# Autodesk Inventor assembly: Drone_rotor_arm_assembly
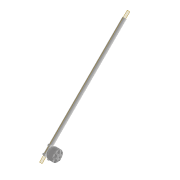
[picture p0: Inventor's stored thumbnail of the model, 180x180]
Saved by Autodesk Inventor 2022 (Build 260153000, 153)
## iProperties
Created: 2022-04-28
Part Number: Drone_rotor_arm_assembly
Document SubType Name: Assembly
Designer: dell
Author: dell
## Documents named in this file (6)
- D:\xxxx\Uni\Part IV\MECHENG_700\Part_IV_project_CAD\Bird_skeleton_prototypes\Bird_wing_10_large_V1\Drone_rotor_arm_assembly.iam
- D:\xxxx\Uni\Part IV\MECHENG_700\Part_IV_project_CAD\Bird_skeleton_prototypes\Wing_drone_V1\T-Motor MN3110.iam
- D:\xxxx\Uni\Part IV\MECHENG_700\Part_IV_project_CAD\Bird_skeleton_prototypes\Wing_drone_V1\CF_tube_12mm.ipt
- D:\xxxx\Uni\Part IV\MECHENG_700\Part_IV_project_CAD\Bird_skeleton_prototypes\Wing_drone_V1\Motor_mount_plate.ipt
- D:\xxxx\Uni\Part IV\MECHENG_700\Part_IV_project_CAD\Bird_skeleton_prototypes\Wing_drone_V1\Motor_mount_clamp_p2.ipt
- D:\xxxx\Uni\Part IV\MECHENG_700\Part_IV_project_CAD\Bird_skeleton_prototypes\Wing_drone_V1\Motor_mount_clamp_p1.ipt
## Components (7 placed, 5 different names)
1. T-Motor MN3110:1 [sub-assembly] — Mate:4, Mate:5, Mate:6
2. CF_tube_12mm:1 — Mate:13, Angle:1, Flush:1
3. Motor_mount_plate:1 — Mate:4, Mate:5, Mate:6, Mate:7, Mate:8, Mate:9, Angle:1, Mate:14, Mate:15, Mate:16, Mate:18, Mate:19
4. Motor_mount_clamp_p2:2 — Mate:7, Mate:8, Mate:9, Mate:10, Mate:11, Mate:12, Mate:13
5. Motor_mount_clamp_p1:1 — Mate:10, Mate:11, Mate:12, Flush:1
6. Motor_mount_clamp_p2:3 — Mate:14, Mate:15, Mate:16, Mate:17
7. Motor_mount_clamp_p1:2 — Mate:17, Mate:18, Mate:19
## Relationships (18: Mate 16, Angle 1, Flush 1)
- Mate:4: T-Motor MN3110:1 ↔ Motor_mount_plate:1
- Mate:5: T-Motor MN3110:1 ↔ Motor_mount_plate:1
- Mate:6: T-Motor MN3110:1 ↔ Motor_mount_plate:1
- Mate:7: Motor_mount_plate:1 ↔ Motor_mount_clamp_p2:2
- Mate:8: Motor_mount_plate:1 ↔ Motor_mount_clamp_p2:2
- Mate:9: Motor_mount_plate:1 ↔ Motor_mount_clamp_p2:2
- Mate:10: Motor_mount_clamp_p2:2 ↔ Motor_mount_clamp_p1:1
- Mate:11: Motor_mount_clamp_p2:2 ↔ Motor_mount_clamp_p1:1
- Mate:12: Motor_mount_clamp_p2:2 ↔ Motor_mount_clamp_p1:1
- Mate:13: CF_tube_12mm:1 ↔ Motor_mount_clamp_p2:2
- Angle:1 (180 deg): CF_tube_12mm:1 ↔ Motor_mount_plate:1
- Mate:14: Motor_mount_plate:1 ↔ Motor_mount_clamp_p2:3
- Mate:15: Motor_mount_plate:1 ↔ Motor_mount_clamp_p2:3
- Mate:16: Motor_mount_plate:1 ↔ Motor_mount_clamp_p2:3
- Mate:17: Motor_mount_clamp_p2:3 ↔ Motor_mount_clamp_p1:2
- Mate:18: Motor_mount_plate:1 ↔ Motor_mount_clamp_p1:2
- Mate:19: Motor_mount_plate:1 ↔ Motor_mount_clamp_p1:2
- Flush:1: CF_tube_12mm:1 ↔ Motor_mount_clamp_p1:1
